# Autodesk Inventor assembly: Assembly1final
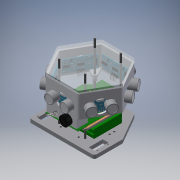
[picture p0: Inventor's stored thumbnail of the model, 180x180]
Saved by Autodesk Inventor 2018 (Build 220112000, 112)
## iProperties
Created: 2017-05-13
Part Number: Assembly1final
Document SubType Name: Assembly
Designer: Vidal Villegas
Author: Vidal Villegas
## Documents named in this file (14)
- C:\Users\Vidal Villegas\Desktop\mp\AssemblyFinalUltimaVersion.iam
- C:\Users\Vidal Villegas\Desktop\mp\base_de_MDF.ipt
- C:\Users\Vidal Villegas\Desktop\mp\tornillo.ipt
- C:\Users\Vidal Villegas\Desktop\mp\base_ultrasonicos.ipt
- C:\Users\Vidal Villegas\Desktop\mp\porta_bateria.ipt
- C:\Users\Vidal Villegas\Desktop\mp\lipo.bateria.ipt
- C:\Users\Vidal Villegas\Desktop\mp\User-Library-HC-SR04.iam
- C:\Users\Vidal Villegas\Desktop\mp\tapa.ipt
- C:\Users\Vidal Villegas\Desktop\mp\porta_switch_y_fusible.ipt
- C:\Users\Vidal Villegas\Desktop\mp\switch\41874.iam
- C:\Users\Vidal Villegas\Desktop\mp\espaciador_largo.ipt
- C:\Users\Vidal Villegas\Desktop\mp\fusible.ipt
- C:\Users\Vidal Villegas\Desktop\mp\espaciador_corto.ipt
- C:\Users\Vidal Villegas\Desktop\mp\placa\PCB2.iam
## Components (27 placed, 13 different names)
1. base_de_MDF:1 — Mate:1, Mate:2, Mate:3, Mate:4, Flush:1, Flush:2, Flush:3, Flush:4, Mate:15
2. tornillo:1 — Mate:1, Flush:4, Mate:19, Mate:28, Cylindrical:5
3. tornillo:2 — Mate:2, Flush:1, Mate:18, Mate:27, Cylindrical:4, Cylindrical:7
4. tornillo:3 — Mate:3, Flush:2, Mate:11, Mate:20, Mate:24, Cylindrical:1, Cylindrical:2, Cylindrical:6
5. tornillo:4 — Mate:4, Flush:3, Mate:10, Mate:21, Mate:25, Mate:29, Cylindrical:3
6. base_ultrasonicos:1 — Mate:10, Mate:11, Insert:1, Mate:14, Insert:2, Insert:3, Insert:4, Insert:5, Insert:6, Insert:7, Insert:8, Insert:9, Insert:10, Insert:11, Mate:26
7. lipo.bateria:1 — Mate:15, Flush:6, Flush:7
8. lipo.bateria:2 — Flush:6, Flush:7, Mate:22, Mate:23
9. User-Library-HC-SR04:1 [sub-assembly] — Insert:1, Mate:14
10. User-Library-HC-SR04:2 [sub-assembly] — Insert:4, Insert:9
11. User-Library-HC-SR04:3 [sub-assembly] — Insert:2, Insert:3
12. User-Library-HC-SR04:4 [sub-assembly] — Insert:5, Insert:6
13. User-Library-HC-SR04:5 [sub-assembly] — Insert:7, Insert:8
14. User-Library-HC-SR04:6 [sub-assembly] — Insert:10, Insert:11
15. porta_bateria:3 — Mate:19, Mate:21, Mate:23
16. porta_bateria:4 — Mate:18, Mate:20, Mate:22
17. tapa:1 — Mate:24, Mate:25, Mate:26
18. porta_switch_y_fusible:1 — Insert:12, Angle:1, Mate:27, Mate:28, Insert:13
19. 41874:1 [sub-assembly] — Insert:12, Angle:1
20. espaciador_largo:1 — Mate:29
21. espaciador_largo:2 — Cylindrical:1
22. fusible:2 — Insert:13
23. espaciador_corto:1 — Cylindrical:2
24. espaciador_corto:2 — Cylindrical:3
25. espaciador_corto:3 — Cylindrical:5
26. espaciador_corto:4 — Cylindrical:4
27. PCB2:1 [sub-assembly] — Cylindrical:6, Cylindrical:7
## Relationships (47: Mate 20, Insert 13, CylindricalJoint 7, Flush 6, Angle 1)
- Mate:1: base_de_MDF:1 ↔ tornillo:1
- Mate:2: base_de_MDF:1 ↔ tornillo:2
- Mate:3: base_de_MDF:1 ↔ tornillo:3
- Mate:4: base_de_MDF:1 ↔ tornillo:4
- Flush:1: base_de_MDF:1 ↔ tornillo:2
- Flush:2: base_de_MDF:1 ↔ tornillo:3
- Flush:3: base_de_MDF:1 ↔ tornillo:4
- Flush:4: base_de_MDF:1 ↔ tornillo:1
- Mate:10: tornillo:4 ↔ base_ultrasonicos:1
- Mate:11: tornillo:3 ↔ base_ultrasonicos:1
- Insert:1: base_ultrasonicos:1 ↔ User-Library-HC-SR04:1
- Mate:14: base_ultrasonicos:1 ↔ User-Library-HC-SR04:1
- Insert:2: base_ultrasonicos:1 ↔ User-Library-HC-SR04:3
- Insert:3: base_ultrasonicos:1 ↔ User-Library-HC-SR04:3
- Insert:4: base_ultrasonicos:1 ↔ User-Library-HC-SR04:2
- Insert:5: base_ultrasonicos:1 ↔ User-Library-HC-SR04:4
- Insert:6: base_ultrasonicos:1 ↔ User-Library-HC-SR04:4
- Insert:7: base_ultrasonicos:1 ↔ User-Library-HC-SR04:5
- Insert:8: base_ultrasonicos:1 ↔ User-Library-HC-SR04:5
- Insert:9: base_ultrasonicos:1 ↔ User-Library-HC-SR04:2
- Insert:10: base_ultrasonicos:1 ↔ User-Library-HC-SR04:6
- Insert:11: base_ultrasonicos:1 ↔ User-Library-HC-SR04:6
- Mate:15: base_de_MDF:1 ↔ lipo.bateria:1
- Flush:6: lipo.bateria:1 ↔ lipo.bateria:2
- Flush:7: lipo.bateria:1 ↔ lipo.bateria:2
- Mate:18: tornillo:2 ↔ porta_bateria:4
- Mate:19: tornillo:1 ↔ porta_bateria:3
- Mate:20: tornillo:3 ↔ porta_bateria:4
- Mate:21: tornillo:4 ↔ porta_bateria:3
- Mate:22: lipo.bateria:2 ↔ porta_bateria:4
- Mate:23: lipo.bateria:2 ↔ porta_bateria:3
- Mate:24: tornillo:3 ↔ tapa:1
- Mate:25: tornillo:4 ↔ tapa:1
- Mate:26: base_ultrasonicos:1 ↔ tapa:1
- Insert:12: porta_switch_y_fusible:1 ↔ 41874:1
- Angle:1 (0 deg): porta_switch_y_fusible:1 ↔ 41874:1
- Mate:27: tornillo:2 ↔ porta_switch_y_fusible:1
- Mate:28: tornillo:1 ↔ porta_switch_y_fusible:1
- Mate:29: tornillo:4 ↔ espaciador_largo:1
- Cylindrical:1: tornillo:3 ↔ espaciador_largo:2
- Insert:13: porta_switch_y_fusible:1 ↔ fusible:2
- Cylindrical:2: tornillo:3 ↔ espaciador_corto:1
- Cylindrical:3: tornillo:4 ↔ espaciador_corto:2
- Cylindrical:4: tornillo:2 ↔ espaciador_corto:4
- Cylindrical:5: tornillo:1 ↔ espaciador_corto:3
- Cylindrical:6: tornillo:3 ↔ PCB2:1
- Cylindrical:7: tornillo:2 ↔ PCB2:1
## Named parameters: sa_0 = -1405.71, sa_1 = -2067.36, sa_2 = -4e-13
note: some values were not read from the file. Shown as the stored number, unit unknown: "sa_0", "sa_1", "sa_2".
